# Autodesk Inventor assembly: main_lcd
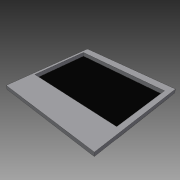
[picture p0: Inventor's stored thumbnail of the model, 180x180]
Saved by Autodesk Inventor 2014 (Build 180170000, 170)
## iProperties
Created: 2014-03-22
Part Number: main_lcd
Document SubType Name: Assembly
Designer: buben
Author: buben
## Documents named in this file (3)
- C:\Users\buben\Documents\GitHub\bacon\inventor files\printer parts\6.5 mm\main_lcd.iam
- C:\Users\buben\Documents\GitHub\bacon\inventor files\printer parts\6.5 mm\main_lcd_front.ipt
- C:\Users\buben\Documents\GitHub\bacon\inventor files\utils\main_lcd_panel.ipt
## Components (2 placed, 2 different names)
1. main_lcd_front:1 — Mate:1, Flush:1, Flush:2
2. main_lcd_panel:1 — Mate:1, Flush:1, Flush:2
## Relationships (3: Flush 2, Mate 1)
- Mate:1: main_lcd_front:1 ↔ main_lcd_panel:1
- Flush:1 (0.5 mm): main_lcd_front:1 ↔ main_lcd_panel:1
- Flush:2 (0.5 mm): main_lcd_front:1 ↔ main_lcd_panel:1
